# Autodesk Inventor assembly: Idler Assembly
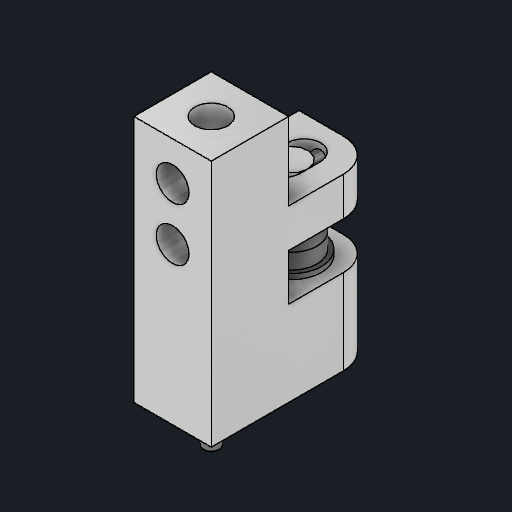
[picture p0: Inventor's stored thumbnail of the model, 512x512]
Saved by Autodesk Inventor 2026.1 (Build 301233020, 233B)
## iProperties
Created: 2025-05-27
Part Number: Idler Assembly
Document SubType Name: Assembly
Designer: Joshua Eah
Author: Joshua Eah
## Documents named in this file (9)
- C:\Users\JoshuaEah\Documents\GitHub\Voron-0\CAD\Tulip - Machined Parts\Idlers\B Idler (Tulip) Assembly.iam
- C:\Users\JoshuaEah\Documents\GitHub\Voron-0\CAD\Master Assembly\Hardware\F623 Stack.iam
- C:\Users\JoshuaEah\Documents\GitHub\Voron-0\CAD\Tulip - Machined Parts\Idlers\Bearing Nut.ipt
- C:\Users\JoshuaEah\Documents\GitHub\Voron-0\CAD\Master Assembly\Hardware\3x12 Pin.ipt
- C:\Users\JoshuaEah\Documents\GitHub\Voron-0\CAD\Tulip - Machined Parts\Idlers\B Idler (Tulip).ipt
- C:\Users\JoshuaEah\Documents\GitHub\Voron-0\CAD\Master Assembly\Hardware\M3x20 SHCS.ipt
- C:\Users\JoshuaEah\Documents\GitHub\Voron-0\CAD\Master Assembly\Hardware\M3x10 BHCS.ipt
- C:\Users\JoshuaEah\Documents\GitHub\Voron-0\CAD\Master Assembly\Hardware\M3x30 BHCS.ipt
- C:\Users\JoshuaEah\Documents\GitHub\Voron-0\CAD\Master Assembly\Hardware\M3x14 Grub Screw.ipt
## Components (9 placed, 8 different names)
1. B Idler (Tulip):1 — Mate:8, Mate:9, Insert:3, Insert:4, Insert:5, Mate:10, Tangent:1
2. Bearing Nut:1 — Mate:6, Insert:2, Mate:8
3. Bearing Nut:2 — Mate:5, Insert:1, Mate:9
4. 3x12 Pin:1 — Mate:5, Mate:6, Insert:1
5. F623 Stack:1 [sub-assembly] — Insert:2
6. M3x20 SHCS:1 — Insert:3
7. M3x10 BHCS:1 — Insert:4
8. M3x30 BHCS:1 — Insert:5
9. M3x14 Grub Screw:1 — Mate:10, Tangent:1
## Relationships (11: Mate 5, Insert 5, Tangent 1)
- Mate:5: Bearing Nut:2 ↔ 3x12 Pin:1
- Mate:6: Bearing Nut:1 ↔ 3x12 Pin:1
- Insert:1: Bearing Nut:2 ↔ 3x12 Pin:1
- Insert:2: Bearing Nut:1 ↔ F623 Stack:1
- Mate:8: B Idler (Tulip):1 ↔ Bearing Nut:1
- Mate:9: B Idler (Tulip):1 ↔ Bearing Nut:2
- Insert:3: B Idler (Tulip):1 ↔ M3x20 SHCS:1
- Insert:4: B Idler (Tulip):1 ↔ M3x10 BHCS:1
- Insert:5: B Idler (Tulip):1 ↔ M3x30 BHCS:1
- Mate:10: B Idler (Tulip):1 ↔ M3x14 Grub Screw:1
- Tangent:1: B Idler (Tulip):1 ↔ M3x14 Grub Screw:1
